# Autodesk Inventor assembly: SPE37V1 Cierre Superior
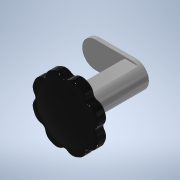
[picture p0: Inventor's stored thumbnail of the model, 180x180]
Saved by Autodesk Inventor 2021.2 (Build 252289000, 289)
## iProperties
Created: 2026-08-18
Part Number: SPE37V1 Cierre Superior
Document SubType Name: Assembly
Designer: nelso
Author: nelso
## Documents named in this file (4)
- C:\Users\nelso\Desktop\Soporte-Paciente-Espinografia\Workspace\SPE37V1 Cierre Superior.iam
- C:\Users\nelso\Desktop\Soporte-Paciente-Espinografia\Workspace\SP34V1 Pomo Cierre.ipt
- C:\Users\nelso\Desktop\Soporte-Paciente-Espinografia\Workspace\SP35V1 Vastago Cierre.ipt
- C:\Users\nelso\Desktop\Soporte-Paciente-Espinografia\Workspace\SP36V1 Traba Cierre.ipt
## Components (3 placed, 3 different names)
1. SP34V1 Pomo Cierre:1 — Mate:1, Mate:3
2. SP35V1 Vastago Cierre:1 — Mate:1, Mate:2, Mate:3, Mate:4
3. SP36V1 Traba Cierre:1 — Mate:2, Mate:4
## Relationships (4: Mate 4)
- Mate:1: SP34V1 Pomo Cierre:1 ↔ SP35V1 Vastago Cierre:1
- Mate:2: SP35V1 Vastago Cierre:1 ↔ SP36V1 Traba Cierre:1
- Mate:3 (-4 mm): SP34V1 Pomo Cierre:1 ↔ SP35V1 Vastago Cierre:1
- Mate:4: SP35V1 Vastago Cierre:1 ↔ SP36V1 Traba Cierre:1
